# Autodesk Inventor assembly: Wheel Assembled
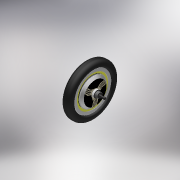
[picture p0: Inventor's stored thumbnail of the model, 180x180]
Saved by Autodesk Inventor 2020 (Build 240168000, 168)
## iProperties
Created: 2019-05-15
Part Number: Wheel Assembled
Document SubType Name: Assembly
Designer: Administrator
Mass: 4808.66 g
Surface Area: 10608.8 cm^2
Volume: 3129.44 cm^3
Density: 1.53659 g/cm^3
Title: Wheel Assembled v49
Author: Administrator
## Documents named in this file (10)
- C:\Users\chitl\Desktop\OneWheel\Wheel Assembled\Wheel Assembled.iam
- C:\Users\chitl\Desktop\OneWheel\Wheel Assembled\Wheel\Tyre.ipt
- C:\Users\chitl\Desktop\OneWheel\Wheel Assembled\Wheel\Axle.ipt
- C:\Users\chitl\Desktop\OneWheel\Wheel Assembled\Wheel\Hub.ipt
- C:\Users\chitl\Desktop\OneWheel\Wheel Assembled\Wheel\Design (5).ipt
- C:\Users\chitl\Desktop\OneWheel\Wheel Assembled\Wheel\Design (4).ipt
- C:\Users\chitl\Desktop\OneWheel\Wheel Assembled\Wheel\Design.ipt
- C:\Users\chitl\Desktop\OneWheel\Wheel Assembled\Wheel\Design (3).ipt
- C:\Users\chitl\Desktop\OneWheel\Wheel Assembled\Wheel\Design (2).ipt
- C:\Users\chitl\Desktop\OneWheel\Wheel Assembled\Wheel\Design (1).ipt
## Components (9 placed, 9 different names)
1. Hub:1 — Insert:1, Mate:2
2. Tyre:1 — Insert:1
3. Axle:1 — Mate:2
4. Design (5):1
5. Design (4):1
6. Design:1
7. Design (3):1
8. Design (2):1
9. Design (1):1
## Relationships (2: Insert 1, Mate 1)
- Insert:1: Hub:1 ↔ Tyre:1
- Mate:2: Hub:1 ↔ Axle:1
